# Autodesk Inventor assembly: rapid-prototype
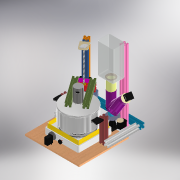
[picture p0: Inventor's stored thumbnail of the model, 180x180]
Saved by Autodesk Inventor 2020 (Build 240168000, 168)
## iProperties
Created: 2020-06-18
Part Number: rapid-prototype
Document SubType Name: Assembly
Designer: pc-konvi
Author: pc-konvi
## Documents named in this file (29)
- C:\Users\pc-konvi\Documents\Lobola\open_source_scrabble\lobola - rapid prototype\rapid-prototype.iam
- C:\Users\pc-konvi\Documents\Lobola\open_source_scrabble\lobola - rapid prototype\Hot Plate.ipt
- C:\Users\pc-konvi\Documents\Lobola\open_source_scrabble\lobola - rapid prototype\Pot.ipt
- C:\Users\pc-konvi\Documents\Lobola\open_source_scrabble\lobola - rapid prototype\heat shield\Heat_shield.iam
- C:\Users\pc-konvi\Documents\Lobola\open_source_scrabble\lobola - rapid prototype\LeadScrewMotor.iam
- C:\Users\pc-konvi\Documents\Lobola\open_source_scrabble\lobola - rapid prototype\bracket.ipt
- C:\Users\pc-konvi\Documents\Lobola\open_source_scrabble\lobola - rapid prototype\trail.ipt
- C:\Users\pc-konvi\Documents\Lobola\open_source_scrabble\lobola - rapid prototype\lid_assembly.iam
- C:\Users\pc-konvi\Documents\Lobola\open_source_scrabble\lobola - rapid prototype\trail_support.ipt
- C:\Users\pc-konvi\Documents\Lobola\open_source_scrabble\lobola - rapid prototype\LeadScrewNut.ipt
- C:\Users\pc-konvi\Documents\Lobola\open_source_scrabble\lobola - rapid prototype\screw_bracket.ipt
- C:\Users\pc-konvi\Documents\Lobola\open_source_scrabble\lobola - rapid prototype\roller.iam
- C:\Users\pc-konvi\Documents\Lobola\open_source_scrabble\lobola - rapid prototype\mixer.iam
- C:\Users\pc-konvi\Documents\Lobola\open_source_scrabble\lobola - rapid prototype\feed.iam
- C:\Users\pc-konvi\Documents\Lobola\open_source_scrabble\lobola - rapid prototype\pin_sleeve.ipt
- C:\Users\pc-konvi\Documents\Lobola\open_source_scrabble\lobola - rapid prototype\servo_motor.ipt
- C:\Users\pc-konvi\Documents\Lobola\open_source_scrabble\lobola - rapid prototype\feed_gear_assembly\Design Accelerator\Spur Gear11.ipt
- C:\Users\pc-konvi\Documents\Lobola\open_source_scrabble\lobola - rapid prototype\servo_pulley.ipt
- C:\Users\pc-konvi\Documents\Lobola\open_source_scrabble\lobola - rapid prototype\stove_pulley.ipt
- C:\Users\pc-konvi\Documents\Lobola\open_source_scrabble\lobola - rapid prototype\flour_duct.ipt
- C:\Users\pc-konvi\Documents\Lobola\open_source_scrabble\lobola - rapid prototype\silo.ipt
- C:\Users\pc-konvi\Documents\Lobola\open_source_scrabble\lobola - rapid prototype\silo_adapter.ipt
- C:\Users\pc-konvi\Documents\Lobola\open_source_scrabble\lobola - rapid prototype\silo_support.ipt
- C:\Users\pc-konvi\Documents\Lobola\open_source_scrabble\lobola - rapid prototype\wooden_base.ipt
- C:\Users\pc-konvi\Documents\Lobola\open_source_scrabble\lobola - rapid prototype\base_pole.ipt
- C:\Users\pc-konvi\Documents\Lobola\open_source_scrabble\lobola - rapid prototype\pot_antispin.ipt
- C:\Users\pc-konvi\Documents\Lobola\open_source_scrabble\lobola - rapid prototype\base_connector.ipt
- C:\Users\pc-konvi\Documents\Lobola\open_source_scrabble\lobola - rapid prototype\pole_supoort_1.ipt
- C:\Users\pc-konvi\Documents\Lobola\open_source_scrabble\lobola - rapid prototype\pole_supoort_2.ipt
## Components (32 placed, 32 different names)
1. Hot Plate — Mate:1, Flush:1, Flush:2, pot-stove, Mate:7, Mate:8, Mate:9, Mate:27, Mate:28, Flush:12, Angle:3, Mate:34, Mate:36, Flush:16, Mate:48, Mate:52, Mate:53, Flush:24
2. Pot — pot-center, pot-align, pot-stove, Flush:11
3. Heat_shield [sub-assembly] — Mate:8, Mate:9, Angle:1, Flush:3, Mate:10
4. roller [sub-assembly] — Flush:9, Mate:24, Flush:10
5. LeadScrewMotor [sub-assembly] — Mate:7, Flush:3, Mate:10, Mate:12, Mate:14
6. lid_assembly [sub-assembly] — Mate:17, Mate:18, Mate:20, Mate:21, Flush:10, Mate:25, Mate:26, temporary
7. mixer [sub-assembly] — Mate:25, Mate:26
8. feed [sub-assembly] — Flush:11, Mate:27, Mate:28, temporary, Mate:29, Flush:13, Mate:39, Mate:40, Mate:47
9. btm_bracket — Mate:11, Mate:13, Mate:14, Flush:4, Mate:15, Mate:16, Flush:6
10. top_bracket — Mate:11, Mate:12, Mate:13, Flush:4, Mate:18, Mate:22, Mate:23, Angle:2
11. trail_pole — Mate:15, Mate:16, Flush:6, Mate:19, Flush:7, Flush:8, Flush:9, Mate:24
12. trail_pole_support — Mate:19, Flush:7, Flush:8, Flush:15, Tangent:2, Flush:28, Mate:59, Mate:60, Flush:29
13. screw_nut — Mate:20, Mate:21
14. screw_bracket — Mate:22, Mate:23, Angle:2
15. pin_sleeve — Mate:29, Flush:12, Angle:3, Mate:31, Angle:4, Mate:33, Angle:6, Flush:19
16. feed_servo_motor — Mate:30, Mate:31, Angle:4, Mate:32, Mate:33, Flush:18
17. feed_servo_gear — Mate:30, Flush:13, Mate:32
18. stove_servo_motor — Mate:35, Mate:38, Angle:5, Mate:49
19. servo_pulley — Flush:14, Mate:35, Mate:37, Mate:38
20. stove_pulley — Mate:34, Flush:14, Mate:36, Mate:37
21. flour_duct — Mate:39, Mate:40, Mate:45, Mate:46
22. silo:1 — Mate:41, Mate:42, Mate:46, Angle:6
23. silo_adapter — Mate:41, Mate:42, Mate:45, Mate:47
24. silo_support — Flush:15, Flush:16, Mate:48, Flush:17, Mate:50
25. wooden_base:1 — Flush:17, Flush:18, Flush:19, Mate:49, Flush:21, Mate:54, Mate:56
26. base_pole — Mate:50, Flush:21, Mate:55, Flush:27, Mate:58
27. pot_antispin_right — Mate:51, Flush:22, Mate:52, Flush:23, Mate:57
28. pot_antispin_left — Mate:51, Flush:22, Flush:23, Mate:53, Mate:54, Flush:24
29. base_connector_right — Flush:25, Flush:26, Mate:55, Mate:56, Mate:57, Flush:27
30. base_connector_left — Flush:25, Flush:26, Tangent:2, Mate:61
31. pole_supoort_1:1 — Mate:58, Flush:28, Mate:59
32. pole_supoort_2:1 — Mate:60, Flush:29, Mate:61
## Relationships (92: Mate 57, Flush 27, Angle 6, Tangent 2)
- Mate:1: Hot Plate
- Flush:1: Hot Plate
- Flush:2: Hot Plate
- pot-center [Mate]: Pot
- pot-align [Mate]: Pot
- pot-stove [Mate]: Hot Plate ↔ Pot
- Mate:7: Hot Plate ↔ LeadScrewMotor
- Mate:8: Hot Plate ↔ Heat_shield
- Mate:9: Hot Plate ↔ Heat_shield
- Angle:1 (0 deg): Heat_shield
- Flush:3 (-2 mm): Heat_shield ↔ LeadScrewMotor
- Mate:10 (2 mm): Heat_shield ↔ LeadScrewMotor
- Mate:11: btm_bracket ↔ top_bracket
- Mate:12: LeadScrewMotor ↔ top_bracket
- Mate:13 (318 mm): btm_bracket ↔ top_bracket
- Mate:14: LeadScrewMotor ↔ btm_bracket
- Flush:4: btm_bracket ↔ top_bracket
- Mate:15: btm_bracket ↔ trail_pole
- Mate:16: btm_bracket ↔ trail_pole
- Flush:6: btm_bracket ↔ trail_pole
- Mate:17: lid_assembly
- Mate:18: lid_assembly ↔ top_bracket
- Mate:19: trail_pole ↔ trail_pole_support
- Flush:7: trail_pole ↔ trail_pole_support
- Flush:8: trail_pole ↔ trail_pole_support
- Mate:20: lid_assembly ↔ screw_nut
- Mate:21: lid_assembly ↔ screw_nut
- Mate:22: top_bracket ↔ screw_bracket
- Mate:23: top_bracket ↔ screw_bracket
- Angle:2 (50 deg): top_bracket ↔ screw_bracket
- Flush:9: roller ↔ trail_pole
- Mate:24: roller ↔ trail_pole
- Flush:10: roller ↔ lid_assembly
- Mate:25: lid_assembly ↔ mixer
- Mate:26 (-10 mm): lid_assembly ↔ mixer
- Flush:11 (83 mm): Pot ↔ feed
- Mate:27 (-35 mm): Hot Plate ↔ feed
- Mate:28 (35 mm): Hot Plate ↔ feed
- temporary [Tangent]: lid_assembly ↔ feed
- Mate:29: feed ↔ pin_sleeve
- Flush:12: Hot Plate ↔ pin_sleeve
- Angle:3 (0 deg): Hot Plate ↔ pin_sleeve
- Mate:30: feed_servo_motor ↔ feed_servo_gear
- Flush:13: feed ↔ feed_servo_gear
- Mate:31 (50 mm): pin_sleeve ↔ feed_servo_motor
- Angle:4 (-90 deg): pin_sleeve ↔ feed_servo_motor
- Mate:32 (1 mm): feed_servo_motor ↔ feed_servo_gear
- Mate:33: pin_sleeve ↔ feed_servo_motor
- Mate:34: Hot Plate ↔ stove_pulley
- Flush:14: servo_pulley ↔ stove_pulley
- Mate:35: stove_servo_motor ↔ servo_pulley
- Mate:36: Hot Plate ↔ stove_pulley
- Mate:37 (50 mm): servo_pulley ↔ stove_pulley
- Mate:38 (1 mm): stove_servo_motor ↔ servo_pulley
- Angle:5 (0 deg): stove_servo_motor
- Mate:39: feed ↔ flour_duct
- Mate:40 (3 mm): feed ↔ flour_duct
- Mate:41: silo:1 ↔ silo_adapter
- Mate:42: silo:1 ↔ silo_adapter
- Mate:45: flour_duct ↔ silo_adapter
- Mate:46: flour_duct ↔ silo:1
- Mate:47: feed ↔ silo_adapter
- Angle:6 (90 deg): pin_sleeve ↔ silo:1
- Flush:15: trail_pole_support ↔ silo_support
- Flush:16 (10 mm): Hot Plate ↔ silo_support
- Mate:48 (86.5 mm): Hot Plate ↔ silo_support
- Flush:17: silo_support ↔ wooden_base:1
- Flush:18 (-35.3 mm): feed_servo_motor ↔ wooden_base:1
- Flush:19 (15 mm): pin_sleeve ↔ wooden_base:1
- Mate:49: stove_servo_motor ↔ wooden_base:1
- Mate:50: silo_support ↔ base_pole
- Flush:21: wooden_base:1 ↔ base_pole
- Mate:51: pot_antispin_right ↔ pot_antispin_left
- Flush:22: pot_antispin_right ↔ pot_antispin_left
- Mate:52: Hot Plate ↔ pot_antispin_right
- Flush:23: pot_antispin_right ↔ pot_antispin_left
- Mate:53: Hot Plate ↔ pot_antispin_left
- Mate:54: wooden_base:1 ↔ pot_antispin_left
- Flush:24 (55 mm): Hot Plate ↔ pot_antispin_left
- Flush:25: base_connector_right ↔ base_connector_left
- Flush:26: base_connector_right ↔ base_connector_left
- Mate:55: base_pole ↔ base_connector_right
- Mate:56: wooden_base:1 ↔ base_connector_right
- Mate:57: pot_antispin_right ↔ base_connector_right
- Tangent:2: trail_pole_support ↔ base_connector_left
- Flush:27: base_pole ↔ base_connector_right
- Mate:58: base_pole ↔ pole_supoort_1:1
- Flush:28: trail_pole_support ↔ pole_supoort_1:1
- Mate:59: trail_pole_support ↔ pole_supoort_1:1
- Mate:60: trail_pole_support ↔ pole_supoort_2:1
- Flush:29: trail_pole_support ↔ pole_supoort_2:1
- Mate:61: base_connector_left ↔ pole_supoort_2:1
